# Autodesk Inventor assembly: Stator_Assembly
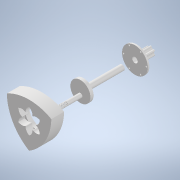
[picture p0: Inventor's stored thumbnail of the model, 180x180]
Saved by Autodesk Inventor 2021 (Build 250183000, 183)
## iProperties
Created: 2021-03-28
Part Number: Stator_Assembly
Document SubType Name: Assembly
Designer: lucia
Author: lucia
## Documents named in this file (4)
- E:\Documents\Inventor\Fixed Rotor Wankel Engine\Assemblies\Stator_Assembly.iam
- E:\Documents\Inventor\Fixed Rotor Wankel Engine\Parts\Rotor_Mount.ipt
- E:\Documents\Inventor\Fixed Rotor Wankel Engine\Parts\Eccentric_Shaft.ipt
- E:\Documents\Inventor\Fixed Rotor Wankel Engine\Parts\Rotor_Geared_6t_Mountable.ipt
## Components (3 placed, 3 different names)
1. Rotor_Mount:1 — Mate:1, Flush:1, Mate:3, Mate:4, Mate:5, Mate:6
2. Eccentric_Shaft:1 — Mate:3, Mate:4
3. Rotor_Geared_6t_Mountable:1 — Mate:5, Mate:6
## Relationships (7: Mate 6, Flush 1)
- Mate:1: Rotor_Mount:1
- Mate:2
- Flush:1: Rotor_Mount:1
- Mate:3 (203.2 mm): Rotor_Mount:1 ↔ Eccentric_Shaft:1
- Mate:4: Rotor_Mount:1 ↔ Eccentric_Shaft:1
- Mate:5 (381 mm): Rotor_Mount:1 ↔ Rotor_Geared_6t_Mountable:1
- Mate:6: Rotor_Mount:1 ↔ Rotor_Geared_6t_Mountable:1
